# Autodesk Inventor assembly: leg_Left_coxa_ass
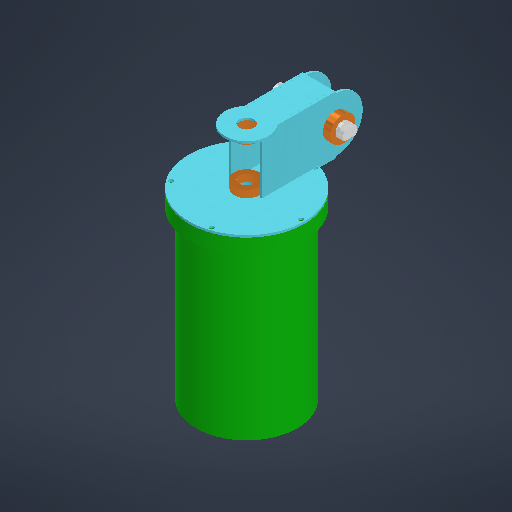
[picture p0: Inventor's stored thumbnail of the model, 512x512]
Saved by Autodesk Inventor 2026 (Build 300175000, 175)
## iProperties
Created: 2026-04-25
Part Number: leg_Left_coxa_ass
Document SubType Name: Assembly
Designer: user
Mass: 4348.06 g
Surface Area: 3136.57 cm^2
Volume: 2916.5 cm^3
Density: 1.49085 g/cm^3
Author: user
## Documents named in this file (7)
- C:\Users\user\Documents\spider_metal\leg_coxa\leg_Left_coxa_ass.iam
- C:\Users\user\Documents\spider_metal\leg_coxa\femur_motor_steel.ipt
- C:\Users\user\Documents\spider_metal\leg_coxa\coxa_support_steel.ipt
- C:\Users\user\Documents\spider_metal\leg_coxa\coxa_upper_steel.ipt
- C:\Users\user\Documents\spider_metal\leg_coxa\shaft_coxa.ipt
- C:\Users\user\Documents\spider_metal\body_parts\motor_mass.ipt
- C:\Users\user\Documents\spider_metal\body_parts\bearing_mass.ipt
## Components (10 placed, 6 different names)
1. femur_motor_steel:1 — Жесткий:4, Жесткий:5, С поворотом:1, С поворотом:2, С поворотом:3
2. coxa_support_steel:1 — Жесткий:7, С поворотом:4
3. coxa_upper_steel:1 — Жесткий:5, С поворотом:6
4. coxa_upper_steel:2 — Жесткий:4, Жесткий:6, Жесткий:7, С поворотом:5
5. shaft_coxa:1 — Жесткий:6
6. motor_mass:1 — С поворотом:1, С поворотом:2
7. bearing_mass:1 — С поворотом:5
8. bearing_mass:2 — С поворотом:6
9. bearing_mass:3 — С поворотом:4
10. bearing_mass:4 — С поворотом:3
## Relationships (10: RevoluteJoint 6, WeldJoint 4)
- Жесткий:4 [WeldJoint]: femur_motor_steel:1 ↔ coxa_upper_steel:2
- Жесткий:5 [WeldJoint]: femur_motor_steel:1 ↔ coxa_upper_steel:1
- Жесткий:6 [WeldJoint] (-20 mm): coxa_upper_steel:2 ↔ shaft_coxa:1
- С поворотом:1 [RevoluteJoint]: femur_motor_steel:1 ↔ motor_mass:1
- С поворотом:2 [RevoluteJoint]: femur_motor_steel:1 ↔ motor_mass:1
- Жесткий:7 [WeldJoint]: coxa_support_steel:1 ↔ coxa_upper_steel:2
- С поворотом:3 [RevoluteJoint]: femur_motor_steel:1 ↔ bearing_mass:4
- С поворотом:4 [RevoluteJoint]: coxa_support_steel:1 ↔ bearing_mass:3
- С поворотом:5 [RevoluteJoint]: coxa_upper_steel:2 ↔ bearing_mass:1
- С поворотом:6 [RevoluteJoint]: coxa_upper_steel:1 ↔ bearing_mass:2
## Named parameters: length_coxa = 180 mm, width_coxa = 74 mm, hight_coxa = 40 mm
